# Autodesk Inventor assembly: PowerSwitchBoardAssembly
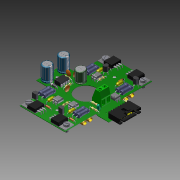
[picture p0: Inventor's stored thumbnail of the model, 180x180]
Saved by Autodesk Inventor 2012 (Build 160160000, 160)
## iProperties
Created: 2014-07-11
Part Number: PowerSwitchBoardAssembly
Document SubType Name: Assembly
Designer: Anon
Author: Anon
## Documents named in this file (5)
- D:\Dropbox\Courses\GP\Inventor\dronestructure\electronics\powerswitch\PowerSwitchBoardAssembly.iam
- D:\Dropbox\Courses\GP\Inventor\dronestructure\electronics\powerswitch\PowerSwitchBoard.iam
- D:\Dropbox\Courses\GP\Inventor\dronestructure\electronics\powerswitch\PowerSwitchSpacer.ipt
- C:\Users\Anon\Documents\Inventor\Content Center Files\R2012\en-US\ISO 1207(2)\ISO 1207 - M3 x 6.ipt
- C:\Users\Anon\Documents\Inventor\Content Center Files\R2012\en-US\ISO 4035(1)\ISO 4035 - M3DIN EN.ipt
## Components (13 placed, 4 different names)
1. PowerSwitchBoard:1 [sub-assembly] — Mate:1, Mate:2, Mate:3, Mate:4, Mate:5, Mate:6, Mate:7, Mate:8, Mate:9, Mate:11, Mate:12, Mate:14, Mate:15, Mate:16, Mate:18, Mate:20, Mate:21, Mate:22, Mate:23, Mate:24
2. PowerSwitchSpacer:1 — Mate:3, Mate:4
3. PowerSwitchSpacer:2 — Mate:1, Mate:2
4. PowerSwitchSpacer:3 — Mate:5, Mate:6
5. PowerSwitchSpacer:4 — Mate:7, Mate:8
6. ISO 1207 M3 x 6:1 — Mate:9, Mate:10, Mate:23
7. ISO 1207 M3 x 6:2 — Mate:15, Mate:17, Mate:22
8. ISO 1207 M3 x 6:3 — Mate:12, Mate:13, Mate:24
9. ISO 1207 M3 x 6:4 — Mate:16, Mate:19, Mate:21
10. DIN EN 24035 M3:1 — Mate:13, Mate:14
11. DIN EN 24035 M3:2 — Mate:17, Mate:18
12. DIN EN 24035 M3:3 — Mate:10, Mate:11
13. DIN EN 24035 M3:4 — Mate:19, Mate:20
## Relationships (24: Mate 24)
- Mate:1: PowerSwitchBoard:1 ↔ PowerSwitchSpacer:2
- Mate:2: PowerSwitchBoard:1 ↔ PowerSwitchSpacer:2
- Mate:3: PowerSwitchBoard:1 ↔ PowerSwitchSpacer:1
- Mate:4: PowerSwitchBoard:1 ↔ PowerSwitchSpacer:1
- Mate:5: PowerSwitchBoard:1 ↔ PowerSwitchSpacer:3
- Mate:6: PowerSwitchBoard:1 ↔ PowerSwitchSpacer:3
- Mate:7: PowerSwitchBoard:1 ↔ PowerSwitchSpacer:4
- Mate:8: PowerSwitchBoard:1 ↔ PowerSwitchSpacer:4
- Mate:9: PowerSwitchBoard:1 ↔ ISO 1207 M3 x 6:1
- Mate:10: ISO 1207 M3 x 6:1 ↔ DIN EN 24035 M3:3
- Mate:11: PowerSwitchBoard:1 ↔ DIN EN 24035 M3:3
- Mate:12: PowerSwitchBoard:1 ↔ ISO 1207 M3 x 6:3
- Mate:13: ISO 1207 M3 x 6:3 ↔ DIN EN 24035 M3:1
- Mate:14: PowerSwitchBoard:1 ↔ DIN EN 24035 M3:1
- Mate:15: PowerSwitchBoard:1 ↔ ISO 1207 M3 x 6:2
- Mate:16: PowerSwitchBoard:1 ↔ ISO 1207 M3 x 6:4
- Mate:17: ISO 1207 M3 x 6:2 ↔ DIN EN 24035 M3:2
- Mate:18: PowerSwitchBoard:1 ↔ DIN EN 24035 M3:2
- Mate:19: ISO 1207 M3 x 6:4 ↔ DIN EN 24035 M3:4
- Mate:20: PowerSwitchBoard:1 ↔ DIN EN 24035 M3:4
- Mate:21: PowerSwitchBoard:1 ↔ ISO 1207 M3 x 6:4
- Mate:22: PowerSwitchBoard:1 ↔ ISO 1207 M3 x 6:2
- Mate:23: PowerSwitchBoard:1 ↔ ISO 1207 M3 x 6:1
- Mate:24: PowerSwitchBoard:1 ↔ ISO 1207 M3 x 6:3
